# Autodesk Inventor assembly: Ensamblaje1
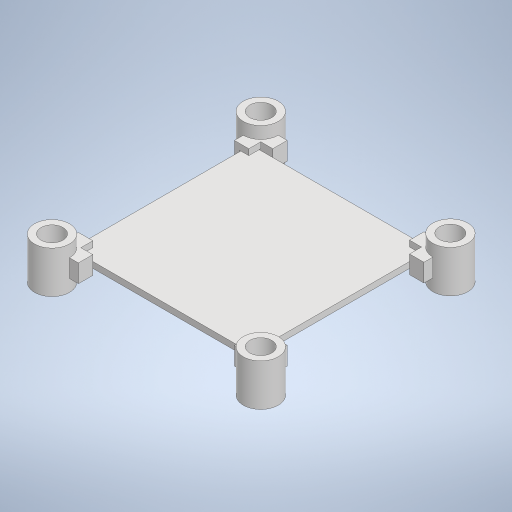
[picture p0: Inventor's stored thumbnail of the model, 512x512]
Saved by Autodesk Inventor 2024 (Build 280153000, 153)
## iProperties
Created: 2023-06-22
Part Number: Ensamblaje1
Document SubType Name: Assembly
Designer: Personal
Author: Personal
## Documents named in this file (3)
- D:\Personal\Documents\GitHub\TDG_ReactionWheelsUnloading\Inventor\EyasSat\Ensamblaje1.iam
- D:\Personal\Documents\GitHub\TDG_ReactionWheelsUnloading\Inventor\EyasSat\Placa.ipt
- D:\Personal\Documents\GitHub\TDG_ReactionWheelsUnloading\Inventor\EyasSat\Sujetador.ipt
## Components (5 placed, 2 different names)
1. Placa:1 — Coincidencia:1, Coincidencia:2, Coincidencia:3, Coincidencia:4, Coincidencia:5, Coincidencia:6, Coincidencia:7, Coincidencia:8
2. Sujetador:1 — Coincidencia:3, Coincidencia:4
3. Sujetador:2 — Coincidencia:1, Coincidencia:2
4. Sujetador:3 — Coincidencia:5, Coincidencia:6
5. Sujetador:4 — Coincidencia:7, Coincidencia:8
## Relationships (8: Mate 8)
- Coincidencia:1 [Mate]: Placa:1 ↔ Sujetador:2
- Coincidencia:2 [Mate]: Placa:1 ↔ Sujetador:2
- Coincidencia:3 [Mate]: Placa:1 ↔ Sujetador:1
- Coincidencia:4 [Mate]: Placa:1 ↔ Sujetador:1
- Coincidencia:5 [Mate]: Placa:1 ↔ Sujetador:3
- Coincidencia:6 [Mate]: Placa:1 ↔ Sujetador:3
- Coincidencia:7 [Mate]: Placa:1 ↔ Sujetador:4
- Coincidencia:8 [Mate]: Placa:1 ↔ Sujetador:4
